# Autodesk Inventor assembly: 2040-2040
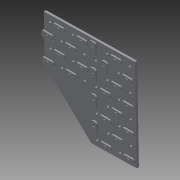
[picture p0: Inventor's stored thumbnail of the model, 180x180]
Saved by Autodesk Inventor 2014 (Build 180170000, 170)
## iProperties
Created: 2014-10-05
Part Number: 2040-2040
Document SubType Name: Assembly
Designer: Matthew
Author: Matthew
## Documents named in this file (3)
- C:\Users\Matthew\Documents\GitHub\CNC Mill\8020\2040-2040.iam
- C:\Users\Matthew\Documents\GitHub\CNC Mill\8020\2040-2040_mounting_plate.ipt
- C:\Users\Matthew\Documents\GitHub\CNC Mill\8020\0.5in_tnut.iam
## Components (25 placed, 2 different names)
1. 2040-2040_mounting_plate:1 — Insert:2, Insert:4, Insert:9, Insert:10, Insert:12, Insert:16, Insert:21, Insert:23, Insert:24, Insert:25, Insert:28, Insert:29, Insert:33, Insert:34, Insert:35, Insert:36, Insert:37, Insert:38, Insert:39, Insert:40, Insert:41, Insert:42, Insert:43, Insert:44
2. 0.5in_tnut:3 [sub-assembly] — Insert:2
3. 0.5in_tnut:6 [sub-assembly] — Insert:4, Flush:1
4. 0.5in_tnut:11 [sub-assembly] — Insert:10
5. 0.5in_tnut:13 [sub-assembly] — Insert:28
6. 0.5in_tnut:14 [sub-assembly] — Insert:33, Flush:2
7. 0.5in_tnut:15 [sub-assembly] — Insert:34
8. 0.5in_tnut:16 [sub-assembly] — Insert:9
9. 0.5in_tnut:20 [sub-assembly] — Insert:36
10. 0.5in_tnut:21 [sub-assembly] — Insert:16
11. 0.5in_tnut:22 [sub-assembly] — Insert:12
12. 0.5in_tnut:27 [sub-assembly] — Insert:35
13. 0.5in_tnut:28 [sub-assembly] — Insert:38
14. 0.5in_tnut:29 [sub-assembly] — Insert:39
15. 0.5in_tnut:31 [sub-assembly] — Insert:44
16. 0.5in_tnut:32 [sub-assembly] — Insert:43
17. 0.5in_tnut:33 [sub-assembly] — Insert:42
18. 0.5in_tnut:34 [sub-assembly] — Insert:41
19. 0.5in_tnut:38 [sub-assembly] — Insert:21
20. 0.5in_tnut:40 [sub-assembly] — Insert:25
21. 0.5in_tnut:42 [sub-assembly] — Insert:23
22. 0.5in_tnut:43 [sub-assembly] — Insert:24, Flush:1
23. 0.5in_tnut:44 [sub-assembly] — Insert:29, Flush:2
24. 0.5in_tnut:45 [sub-assembly] — Insert:37
25. 0.5in_tnut:46 [sub-assembly] — Insert:40
## Relationships (26: Insert 24, Flush 2)
- Insert:2: 2040-2040_mounting_plate:1 ↔ 0.5in_tnut:3
- Insert:4: 2040-2040_mounting_plate:1 ↔ 0.5in_tnut:6
- Insert:9: 2040-2040_mounting_plate:1 ↔ 0.5in_tnut:16
- Insert:10: 2040-2040_mounting_plate:1 ↔ 0.5in_tnut:11
- Insert:12: 2040-2040_mounting_plate:1 ↔ 0.5in_tnut:22
- Insert:16: 2040-2040_mounting_plate:1 ↔ 0.5in_tnut:21
- Insert:21: 2040-2040_mounting_plate:1 ↔ 0.5in_tnut:38
- Insert:23: 2040-2040_mounting_plate:1 ↔ 0.5in_tnut:42
- Insert:24: 2040-2040_mounting_plate:1 ↔ 0.5in_tnut:43
- Insert:25: 2040-2040_mounting_plate:1 ↔ 0.5in_tnut:40
- Insert:28: 2040-2040_mounting_plate:1 ↔ 0.5in_tnut:13
- Insert:29: 2040-2040_mounting_plate:1 ↔ 0.5in_tnut:44
- Insert:33: 2040-2040_mounting_plate:1 ↔ 0.5in_tnut:14
- Insert:34: 2040-2040_mounting_plate:1 ↔ 0.5in_tnut:15
- Flush:1: 0.5in_tnut:6 ↔ 0.5in_tnut:43
- Flush:2: 0.5in_tnut:14 ↔ 0.5in_tnut:44
- Insert:35: 2040-2040_mounting_plate:1 ↔ 0.5in_tnut:27
- Insert:36: 2040-2040_mounting_plate:1 ↔ 0.5in_tnut:20
- Insert:37: 2040-2040_mounting_plate:1 ↔ 0.5in_tnut:45
- Insert:38: 2040-2040_mounting_plate:1 ↔ 0.5in_tnut:28
- Insert:39: 2040-2040_mounting_plate:1 ↔ 0.5in_tnut:29
- Insert:40: 2040-2040_mounting_plate:1 ↔ 0.5in_tnut:46
- Insert:41: 2040-2040_mounting_plate:1 ↔ 0.5in_tnut:34
- Insert:42: 2040-2040_mounting_plate:1 ↔ 0.5in_tnut:33
- Insert:43: 2040-2040_mounting_plate:1 ↔ 0.5in_tnut:32
- Insert:44: 2040-2040_mounting_plate:1 ↔ 0.5in_tnut:31
